# Autodesk Inventor assembly: STM assembly
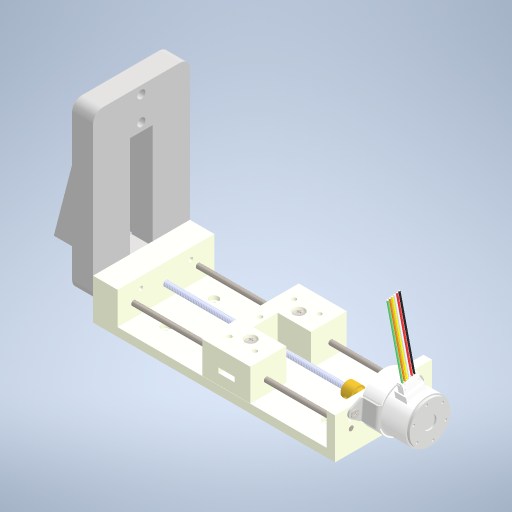
[picture p0: Inventor's stored thumbnail of the model, 512x512]
Saved by Autodesk Inventor 2024 (Build 280153000, 153)
## iProperties
Created: 2023-12-08
Part Number: STM assembly
Document SubType Name: Assembly
Designer: Abdulrahman Riskuwa
Author: Abdulrahman Riskuwa
## Documents named in this file (3)
- C:\Users\Abdulrahman Riskuwa\Documents\FMD 3 Project\STM assembly.iam
- C:\Users\Abdulrahman Riskuwa\Documents\FMD 3 Project\FMDIII.ipt
- C:\Users\Abdulrahman Riskuwa\Documents\FMD 3 Project\stand_less_rough.ipt
## Components (2 placed, 2 different names)
1. FMDIII:1 — Mate:1, Mate:2
2. stand_less_rough:1 — Mate:1, Mate:2
## Relationships (2: Mate 2)
- Mate:1: FMDIII:1 ↔ stand_less_rough:1
- Mate:2: FMDIII:1 ↔ stand_less_rough:1
